# Autodesk Inventor assembly: Main Assembly
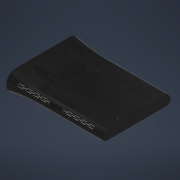
[picture p0: Inventor's stored thumbnail of the model, 180x180]
Saved by Autodesk Inventor 2022 (Build 260153000, 153)
## iProperties
Created: 2021-06-17
Part Number: Main Assembly
Document SubType Name: Assembly
Designer: trl121
Author: trl121
## Documents named in this file (6)
- D:\trl121\Documents\_repositories\RazerBook13Dock\Inventor\Main Assembly.iam
- D:\trl121\Documents\_repositories\RazerBook13Dock\Inventor\Razor Book 13.ipt
- D:\trl121\Documents\_repositories\RazerBook13Dock\Inventor\Bottom Part.ipt
- D:\trl121\Documents\_repositories\RazerBook13Dock\Inventor\Top Part.ipt
- D:\trl121\Documents\_repositories\RazerBook13Dock\Inventor\Mount.ipt
- D:\trl121\Documents\_repositories\RazerBook13Dock\Inventor\USB Clamp.ipt
## Components (6 placed, 5 different names)
1. Razor Book 13:1 — Flush:1, Mate:2
2. Bottom Part:1 — Flush:1, Flush:2, Flush:6, Flush:10, Flush:11, Flush:12, Flush:13, Mate:1, Flush:14, Flush:16, Mate:2
3. Top Part:1 — Flush:2, Flush:6, Flush:10, Flush:18
4. Mount:1 — Flush:11, Flush:12, Flush:18
5. Mount:2 — Flush:13, Mate:1
6. USB Clamp:1 — Flush:14, Flush:16
## Relationships (12: Flush 10, Mate 2)
- Flush:1: Razor Book 13:1 ↔ Bottom Part:1
- Flush:2: Bottom Part:1 ↔ Top Part:1
- Flush:6: Bottom Part:1 ↔ Top Part:1
- Flush:10: Bottom Part:1 ↔ Top Part:1
- Flush:11: Bottom Part:1 ↔ Mount:1
- Flush:12 (0.4064 mm): Bottom Part:1 ↔ Mount:1
- Flush:13: Bottom Part:1 ↔ Mount:2
- Mate:1 (0.2 mm): Bottom Part:1 ↔ Mount:2
- Flush:14: Bottom Part:1 ↔ USB Clamp:1
- Flush:16: Bottom Part:1 ↔ USB Clamp:1
- Flush:18: Top Part:1 ↔ Mount:1
- Mate:2: Razor Book 13:1 ↔ Bottom Part:1
